# Autodesk Inventor assembly: kick
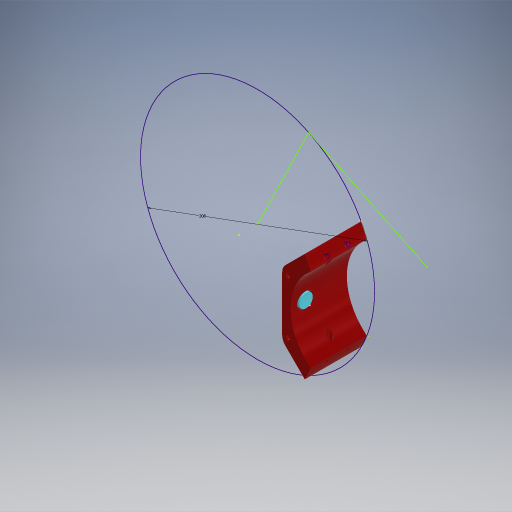
[picture p0: Inventor's stored thumbnail of the model, 512x512]
Saved by Autodesk Inventor 2023 (Build 270158000, 158)
## iProperties
Created: 2025-03-27
Part Number: kick
Document SubType Name: Assembly
Designer: Ivan
Author: Ivan
## Documents named in this file (4)
- C:\!projects\DASH-\3D\Dash-V1\Solenoid\kick.iam
- C:\Users\Ivan\Documents\Inventor\Content Center Files\R2023\ru-RU\ANSI B18.2.4.2M\ANSI B18.2.4.2M - M5x0,8 - 8.ipt
- C:\!projects\DASH-\3D\Dash-V1\Solenoid\kicker.ipt
- C:\!projects\DASH-\3D\Dash-V1\catch_v2.ipt
## Components (3 placed, 3 different names)
1. ANSI B18.2.4.2M M5x0,8:1 — Совмещение:1, Заподлицо:1, Угол:1
2. kicker:1 — Заподлицо:2, Заподлицо:3, Совмещение:2, Заподлицо:4, Заподлицо:5
3. catch_v2:1 — Совмещение:2, Угол:2
## Relationships (9: Flush 5, Mate 2, Angle 2)
- Совмещение:1 [Mate]: ANSI B18.2.4.2M M5x0,8:1
- Заподлицо:1 [Flush]: ANSI B18.2.4.2M M5x0,8:1
- Заподлицо:2 [Flush]: kicker:1
- Заподлицо:3 [Flush]: kicker:1
- Угол:1 [Angle] (0 deg): ANSI B18.2.4.2M M5x0,8:1
- Совмещение:2 [Mate]: kicker:1 ↔ catch_v2:1
- Угол:2 [Angle] (180 deg): catch_v2:1
- Заподлицо:4 [Flush]: kicker:1
- Заподлицо:5 [Flush]: kicker:1
